# Autodesk Inventor assembly: MainAssembly
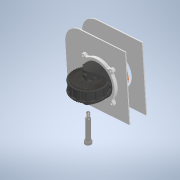
[picture p0: Inventor's stored thumbnail of the model, 180x180]
Saved by Autodesk Inventor 2020 (Build 240168000, 168)
## iProperties
Created: 2019-05-09
Part Number: MainAssembly
Document SubType Name: Assembly
Designer: Connor
Author: Connor
## Documents named in this file (15)
- C:\Users\Connor\Documents\GrabCAD\2019 Robot\Swerve\TorqyoDrift\MainAssembly.iam
- C:\Users\Connor\Documents\GrabCAD\2019 Robot\Imported Components\Wheels and Hubs\VEX Traction Wheels\TractionWheel 4x1\TractionWheel 4x1.iam
- C:\Users\Connor\Documents\GrabCAD\2019 Robot\Swerve\TorqyoDrift\15t_bevel.ipt
- C:\Users\Connor\Documents\GrabCAD\2019 Robot\Swerve\TorqyoDrift\60t_bevel.ipt
- C:\Users\Connor\Documents\GrabCAD\2019 Robot\Swerve\TorqyoDrift\AlternateRingGearAssembly.iam
- C:\Users\Connor\Documents\GrabCAD\2019 Robot\Swerve\TorqyoDrift\ImportedComponentsPlus\Bearings\SA035XPO.ipt
- C:\Users\Connor\Documents\GrabCAD\2019 Robot\Swerve\TorqyoDrift\CenterColumn.ipt
- C:\Users\Connor\Documents\GrabCAD\2019 Robot\Swerve\TorqyoDrift\SingleBracket.ipt
- C:\Users\Connor\Documents\GrabCAD\2019 Robot\Swerve\TorqyoDrift\ImportedComponentsPlus\Hex Gears\16t_Aluminum_Spur_Gear_20_DP_3_8_Hex_Bore_217-5450.ipt
- C:\Users\Connor\Documents\GrabCAD\2019 Robot\Imported Components\Bearings\Radial_0.25x0.375x0.125.ipt
- C:\Users\Connor\Documents\GrabCAD\2019 Robot\Swerve\TorqyoDrift\DriveShaft.ipt
- C:\Users\Connor\Documents\GrabCAD\2019 Robot\Imported Components\Bearings\Radial_0.25x0.5x0.188.ipt
- C:\Users\Connor\Documents\GrabCAD\2019 Robot\Imported Components\Hardware\Specialty\Shoulder Bolt- 0.5x2.25.ipt
- C:\Users\Connor\Documents\GrabCAD\2019 Robot\Swerve\TorqyoDrift\BottomPlate.ipt
- C:\Users\Connor\Documents\GrabCAD\2019 Robot\Swerve\TorqyoDrift\BearingClamp.ipt
## Components (22 placed, 14 different names)
1. TractionWheel 4x1:1 [sub-assembly] — Mate:1, Mate:2, Mate:3, Mate:4, Mate:5, Mate:6, Mate:24
2. 15t_bevel:1 — Tangent:1, Flush:1, Mate:7, Angle:2, Mate:30, Mate:31, Angle:3
3. 60t_bevel:1 — Mate:4, Mate:5, Mate:6, Tangent:1, Flush:1, Mate:7
4. 15t_bevel:2 — Tangent:2, Mate:9, Flush:2, Mate:27, Mate:32, Angle:4
5. 60t_bevel:2 — Mate:1, Mate:2, Mate:3, Tangent:2, Mate:9, Flush:2
6. AlternateRingGearAssembly:1 [sub-assembly] — Mate:14, Mate:28, Mate:29, Flush:3
7. AlternateRingGearAssembly:2 [sub-assembly] — Mate:14, Mate:29, Flush:4
8. SA035XPO:1 — Mate:25, Mate:26, Mate:28, Mate:33, Mate:34, Mate:49, Mate:50, Mate:51, Mate:52
9. CenterColumn:1 — Mate:33, Mate:34, Mate:35, Mate:42, Mate:43, Mate:44, Mate:45, Mate:53
10. SingleBracket:1 — Mate:24, Mate:25, Mate:26, Angle:2, Mate:27, Mate:35, Mate:36, Mate:37, Mate:38, Mate:39, Mate:48
11. 16t_Aluminum_Spur_Gear_20_DP_3_8_Hex_Bore_217-5450:1 — Mate:30, Mate:31, Flush:3, Angle:3
12. 16t_Aluminum_Spur_Gear_20_DP_3_8_Hex_Bore_217-5450:2 — Mate:32, Flush:4, Angle:4
13. Radial_0.25x0.375x0.125:1 — Mate:36, Mate:37, Mate:40, Mate:41
14. Radial_0.25x0.375x0.125:2 — Mate:38, Mate:39
15. DriveShaft:1 — Mate:40, Mate:41
16. Radial_0.25x0.5x0.188:1 — Mate:44, Mate:45, Mate:46, Mate:47
17. Radial_0.25x0.5x0.188:2 — Mate:42, Mate:43
18. DriveShaft:2 — Mate:46, Mate:47
19. Shoulder Bolt- 0.5x2.25:1 — Mate:48
20. BottomPlate:1 — Mate:49, Mate:50, Mate:54, Flush:5
21. BearingClamp:1 — Mate:51, Mate:52
22. BottomPlate:2 — Mate:53, Mate:54, Flush:5
## Relationships (50: Mate 40, Flush 5, Angle 3, Tangent 2)
- Mate:1: TractionWheel 4x1:1 ↔ 60t_bevel:2
- Mate:2: TractionWheel 4x1:1 ↔ 60t_bevel:2
- Mate:3: TractionWheel 4x1:1 ↔ 60t_bevel:2
- Mate:4: TractionWheel 4x1:1 ↔ 60t_bevel:1
- Mate:5: TractionWheel 4x1:1 ↔ 60t_bevel:1
- Mate:6: TractionWheel 4x1:1 ↔ 60t_bevel:1
- Tangent:1 (2 mm): 15t_bevel:1 ↔ 60t_bevel:1
- Flush:1 (56 mm): 15t_bevel:1 ↔ 60t_bevel:1
- Mate:7: 15t_bevel:1 ↔ 60t_bevel:1
- Tangent:2 (2 mm): 15t_bevel:2 ↔ 60t_bevel:2
- Mate:9 (-56 mm): 15t_bevel:2 ↔ 60t_bevel:2
- Flush:2: 15t_bevel:2 ↔ 60t_bevel:2
- Mate:14: AlternateRingGearAssembly:1 ↔ AlternateRingGearAssembly:2
- Mate:24: TractionWheel 4x1:1 ↔ SingleBracket:1
- Mate:25: SA035XPO:1 ↔ SingleBracket:1
- Mate:26: SA035XPO:1 ↔ SingleBracket:1
- Angle:2 (0 deg): 15t_bevel:1 ↔ SingleBracket:1
- Mate:27: 15t_bevel:2 ↔ SingleBracket:1
- Mate:28: AlternateRingGearAssembly:1 ↔ SA035XPO:1
- Mate:29 (1.5875 mm): AlternateRingGearAssembly:1 ↔ AlternateRingGearAssembly:2
- Mate:30: 15t_bevel:1 ↔ 16t_Aluminum_Spur_Gear_20_DP_3_8_Hex_Bore_217-5450:1
- Mate:31: 15t_bevel:1 ↔ 16t_Aluminum_Spur_Gear_20_DP_3_8_Hex_Bore_217-5450:1
- Flush:3: AlternateRingGearAssembly:1 ↔ 16t_Aluminum_Spur_Gear_20_DP_3_8_Hex_Bore_217-5450:1
- Angle:3 (0 deg): 15t_bevel:1 ↔ 16t_Aluminum_Spur_Gear_20_DP_3_8_Hex_Bore_217-5450:1
- Mate:32: 15t_bevel:2 ↔ 16t_Aluminum_Spur_Gear_20_DP_3_8_Hex_Bore_217-5450:2
- Flush:4: AlternateRingGearAssembly:2 ↔ 16t_Aluminum_Spur_Gear_20_DP_3_8_Hex_Bore_217-5450:2
- Angle:4 (0 deg): 15t_bevel:2 ↔ 16t_Aluminum_Spur_Gear_20_DP_3_8_Hex_Bore_217-5450:2
- Mate:33: SA035XPO:1 ↔ CenterColumn:1
- Mate:34: SA035XPO:1 ↔ CenterColumn:1
- Mate:35: CenterColumn:1 ↔ SingleBracket:1
- Mate:36: SingleBracket:1 ↔ Radial_0.25x0.375x0.125:1
- Mate:37: SingleBracket:1 ↔ Radial_0.25x0.375x0.125:1
- Mate:38: SingleBracket:1 ↔ Radial_0.25x0.375x0.125:2
- Mate:39: SingleBracket:1 ↔ Radial_0.25x0.375x0.125:2
- Mate:40: Radial_0.25x0.375x0.125:1 ↔ DriveShaft:1
- Mate:41: Radial_0.25x0.375x0.125:1 ↔ DriveShaft:1
- Mate:42: CenterColumn:1 ↔ Radial_0.25x0.5x0.188:2
- Mate:43: CenterColumn:1 ↔ Radial_0.25x0.5x0.188:2
- Mate:44: CenterColumn:1 ↔ Radial_0.25x0.5x0.188:1
- Mate:45: CenterColumn:1 ↔ Radial_0.25x0.5x0.188:1
- Mate:46: Radial_0.25x0.5x0.188:1 ↔ DriveShaft:2
- Mate:47: Radial_0.25x0.5x0.188:1 ↔ DriveShaft:2
- Mate:48: SingleBracket:1 ↔ Shoulder Bolt- 0.5x2.25:1
- Mate:49: SA035XPO:1 ↔ BottomPlate:1
- Mate:50: SA035XPO:1 ↔ BottomPlate:1
- Mate:51: SA035XPO:1 ↔ BearingClamp:1
- Mate:52: SA035XPO:1 ↔ BearingClamp:1
- Mate:53: CenterColumn:1 ↔ BottomPlate:2
- Mate:54 (50.8 mm): BottomPlate:1 ↔ BottomPlate:2
- Flush:5: BottomPlate:1 ↔ BottomPlate:2
